# Autodesk Inventor assembly: Байонет со статором
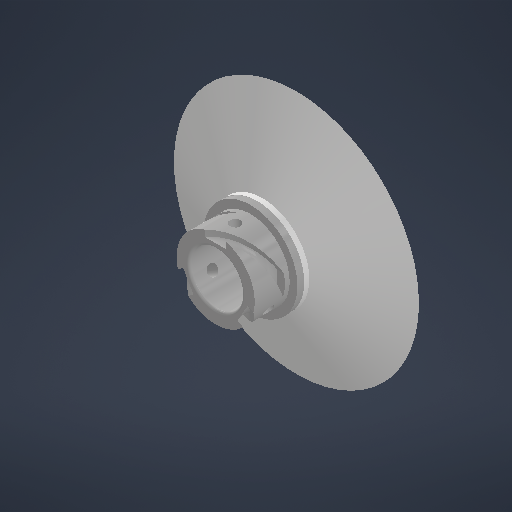
[picture p0: Inventor's stored thumbnail of the model, 512x512]
Saved by Autodesk Inventor 2026 (Build 300175000, 175)
## iProperties
Created: 2025-08-13
Part Number: Байонет со статором
Document SubType Name: Assembly
Designer: kvm13
Author: kvm13
## Documents named in this file (3)
- C:\Users\kvm13\Desktop\MIK-nozzle\3D Форсунка фрикад\Байонет со статором.iam
- C:\Users\kvm13\Desktop\MIK-nozzle\3D Форсунка фрикад\Байонет ванны.ipt
- C:\Users\kvm13\Desktop\MIK-nozzle\3D Форсунка фрикад\Статор диска.ipt
## Components (2 placed, 2 different names)
1. Байонет ванны:1 — С поворотом:1
2. Статор диска:1 — С поворотом:1
## Relationships (1: RevoluteJoint 1)
- С поворотом:1 [RevoluteJoint]: Байонет ванны:1 ↔ Статор диска:1
